# Autodesk Inventor assembly: MQ013xG-ON
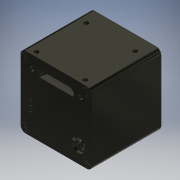
[picture p0: Inventor's stored thumbnail of the model, 180x180]
Saved by Autodesk Inventor 2019 (Build 230136000, 136)
## iProperties
Created: 2012-12-31
Part Number: MQ013xG-ON
Document SubType Name: Assembly
Designer: Brian
Sending System: SIEMENS PLM Software NX 8.5
Preprocessor: ST-DEVELOPER v15
Title: MQ013xG-ON.stp
## Documents named in this file (10)
- C:\Users\Brian\Desktop\designs\MQ013xG-ON\MQ013xG-ON.iam
- C:\Users\Brian\Desktop\designs\MQ013xG-ON\MECH-MQ-MID-013-E2.ipt
- C:\Users\Brian\Desktop\designs\MQ013xG-ON\MECH-MQ-CS-C.ipt
- C:\Users\Brian\Desktop\designs\MQ013xG-ON\MECH-MQ-FRONT.ipt
- C:\Users\Brian\Desktop\designs\MQ013xG-ON\MECH-MQ-REAR.ipt
- C:\Users\Brian\Desktop\designs\MQ013xG-ON\MECH-MQ-LIGHTPIPE.ipt
- C:\Users\Brian\Desktop\designs\MQ013xG-ON\MQ013xG-ON-PCA_MODEL.iam
- C:\Users\Brian\Desktop\designs\MQ013xG-ON\FLT-D25.ipt
- C:\Users\Brian\Desktop\designs\MQ013xG-ON\SROB-M2x10-CUST.ipt
- C:\Users\Brian\Desktop\designs\MQ013xG-ON\SROB-M2x14-CUST.ipt
## Components (17 placed, 17 different names)
1. MECH-MQ-MID-013-E2_1003 — Flush:2, Flush:3, Flush:6, Flush:7, Mate:1, Flush:12, Mate:3, Mate:4
2. MECH-MQ-CS-C_1004 — Flush:1, Flush:2, Flush:4, Flush:5, Flush:6, Mate:2, Mate:3
3. MECH-MQ-FRONT_1005 — Flush:1, Flush:4, Flush:5, Flush:8, Flush:9, Flush:10, Flush:11, Mate:2, Mate:10, Mate:11, Mate:12, Mate:13
4. MECH-MQ-REAR_1006 — Flush:3, Flush:7, Flush:13, Flush:14, Flush:15, Flush:16, Mate:4, Mate:5, Mate:6, Mate:7, Mate:8, Mate:9, Angle:1, Flush:17
5. MECH-MQ-LIGHTPIPE_1007
6. MECH-MQ-LIGHTPIPE_1008
7. MECH-MQ-LIGHTPIPE_1009
8. MQ013xG-ON-PCA_MODEL_1010 [sub-assembly] — Flush:16, Mate:9, Angle:1
9. FLT-D25_1011 — Mate:1, Flush:12
10. SROB-M2x10-CUST_1012 — Flush:13, Mate:5
11. SROB-M2x10-CUST_1013 — Flush:15, Mate:7
12. SROB-M2x10-CUST_1014 — Flush:14, Mate:6
13. SROB-M2x10-CUST_1015 — Mate:8, Flush:17
14. SROB-M2x14-CUST_1016 — Flush:8, Mate:10
15. SROB-M2x14-CUST_1017 — Flush:10, Mate:12
16. SROB-M2x14-CUST_1018 — Flush:9, Mate:13
17. SROB-M2x14-CUST_1019 — Flush:11, Mate:11
## Relationships (31: Flush 17, Mate 13, Angle 1)
- Flush:1: MECH-MQ-CS-C_1004 ↔ MECH-MQ-FRONT_1005
- Flush:2: MECH-MQ-MID-013-E2_1003 ↔ MECH-MQ-CS-C_1004
- Flush:3: MECH-MQ-MID-013-E2_1003 ↔ MECH-MQ-REAR_1006
- Flush:4: MECH-MQ-CS-C_1004 ↔ MECH-MQ-FRONT_1005
- Flush:5: MECH-MQ-CS-C_1004 ↔ MECH-MQ-FRONT_1005
- Flush:6: MECH-MQ-MID-013-E2_1003 ↔ MECH-MQ-CS-C_1004
- Flush:7: MECH-MQ-MID-013-E2_1003 ↔ MECH-MQ-REAR_1006
- Flush:8: MECH-MQ-FRONT_1005 ↔ SROB-M2x14-CUST_1016
- Flush:9: MECH-MQ-FRONT_1005 ↔ SROB-M2x14-CUST_1018
- Flush:10: MECH-MQ-FRONT_1005 ↔ SROB-M2x14-CUST_1017
- Flush:11: MECH-MQ-FRONT_1005 ↔ SROB-M2x14-CUST_1019
- Mate:1: MECH-MQ-MID-013-E2_1003 ↔ FLT-D25_1011
- Flush:12: MECH-MQ-MID-013-E2_1003 ↔ FLT-D25_1011
- Flush:13: MECH-MQ-REAR_1006 ↔ SROB-M2x10-CUST_1012
- Flush:14: MECH-MQ-REAR_1006 ↔ SROB-M2x10-CUST_1014
- Flush:15: MECH-MQ-REAR_1006 ↔ SROB-M2x10-CUST_1013
- Flush:16: MECH-MQ-REAR_1006 ↔ MQ013xG-ON-PCA_MODEL_1010
- Mate:2: MECH-MQ-CS-C_1004 ↔ MECH-MQ-FRONT_1005
- Mate:3: MECH-MQ-MID-013-E2_1003 ↔ MECH-MQ-CS-C_1004
- Mate:4: MECH-MQ-MID-013-E2_1003 ↔ MECH-MQ-REAR_1006
- Mate:5: MECH-MQ-REAR_1006 ↔ SROB-M2x10-CUST_1012
- Mate:6: MECH-MQ-REAR_1006 ↔ SROB-M2x10-CUST_1014
- Mate:7: MECH-MQ-REAR_1006 ↔ SROB-M2x10-CUST_1013
- Mate:8: MECH-MQ-REAR_1006 ↔ SROB-M2x10-CUST_1015
- Mate:9: MECH-MQ-REAR_1006 ↔ MQ013xG-ON-PCA_MODEL_1010
- Angle:1 (90 deg): MECH-MQ-REAR_1006 ↔ MQ013xG-ON-PCA_MODEL_1010
- Flush:17: MECH-MQ-REAR_1006 ↔ SROB-M2x10-CUST_1015
- Mate:10: MECH-MQ-FRONT_1005 ↔ SROB-M2x14-CUST_1016
- Mate:11: MECH-MQ-FRONT_1005 ↔ SROB-M2x14-CUST_1019
- Mate:12: MECH-MQ-FRONT_1005 ↔ SROB-M2x14-CUST_1017
- Mate:13: MECH-MQ-FRONT_1005 ↔ SROB-M2x14-CUST_1018
